# Autodesk Inventor assembly: OpenROV_Dev_Port_EndCap
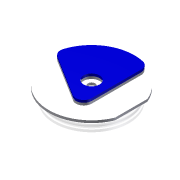
[picture p0: Inventor's stored thumbnail of the model, 180x180]
Saved by Autodesk Inventor 2012 (Build 160160000, 160)
## iProperties
Created: 2012-07-04
Part Number: OpenROV_Dev_Port_EndCap
Document SubType Name: Assembly
Designer: user
Author: user
## Documents named in this file (6)
- C:\Users\user\Desktop\CLEAN ME\OpenROV\openrov-hardware\OpenROV 2.3.2 Dev\OpenROV_Dev_Port_EndCap.iam
- C:\Users\user\Desktop\CLEAN ME\OpenROV\openrov-hardware\OpenROV 2.3.2 Dev\OpenROV_Dev_EndCap_90.ipt
- C:\Users\user\Desktop\CLEAN ME\OpenROV\openrov-hardware\OpenROV 2.3.2 Dev\OpenROV_Dev_EndCap_94.ipt
- C:\Users\user\Desktop\CLEAN ME\OpenROV\openrov-hardware\OpenROV 2.3.2 Dev\OpenROV_Dev_EndCap_108.ipt
- C:\Users\user\Desktop\CLEAN ME\OpenROV\openrov-hardware\OpenROV 2.3.2 Dev\OpenROV_Dev_EndCap_Wire_Guide.ipt
- C:\Users\user\Desktop\CLEAN ME\OpenROV\openrov-hardware\OpenROV 2.3.2 Dev\OpenROV_Dev_EndCap_Wire Guide_Cover.ipt
## Components (8 placed, 5 different names)
1. OpenROV_Dev_EndCap_90:1 — Mate:1, Mate:2, Mate:5, Mate:6, Mate:9, Mate:10
2. OpenROV_Dev_EndCap_90:2 — Mate:3, Mate:4, Mate:7, Mate:8, Mate:11, Mate:12
3. OpenROV_Dev_EndCap_94:1 — Mate:2, Mate:3, Mate:6, Mate:7, Mate:10, Mate:11
4. OpenROV_Dev_EndCap_94:2 — Mate:4, Mate:8, Mate:12, Mate:13, Mate:14, Mate:15
5. OpenROV_Dev_EndCap_94:3 — Mate:1, Mate:5, Mate:9
6. OpenROV_Dev_EndCap_108:1 — Mate:13, Mate:14, Mate:15, Mate:16, Mate:17, Mate:18
7. OpenROV_Dev_EndCap_Wire_Guide:1 — Mate:16, Mate:17, Mate:18, Mate:19, Mate:20, Flush:1
8. OpenROV_Dev_EndCap_Wire Guide_Cover:1 — Mate:19, Mate:20, Flush:1
## Relationships (21: Mate 20, Flush 1)
- Mate:1: OpenROV_Dev_EndCap_90:1 ↔ OpenROV_Dev_EndCap_94:3
- Mate:2: OpenROV_Dev_EndCap_90:1 ↔ OpenROV_Dev_EndCap_94:1
- Mate:3: OpenROV_Dev_EndCap_90:2 ↔ OpenROV_Dev_EndCap_94:1
- Mate:4: OpenROV_Dev_EndCap_90:2 ↔ OpenROV_Dev_EndCap_94:2
- Mate:5: OpenROV_Dev_EndCap_90:1 ↔ OpenROV_Dev_EndCap_94:3
- Mate:6: OpenROV_Dev_EndCap_90:1 ↔ OpenROV_Dev_EndCap_94:1
- Mate:7: OpenROV_Dev_EndCap_90:2 ↔ OpenROV_Dev_EndCap_94:1
- Mate:8: OpenROV_Dev_EndCap_90:2 ↔ OpenROV_Dev_EndCap_94:2
- Mate:9: OpenROV_Dev_EndCap_90:1 ↔ OpenROV_Dev_EndCap_94:3
- Mate:10: OpenROV_Dev_EndCap_90:1 ↔ OpenROV_Dev_EndCap_94:1
- Mate:11: OpenROV_Dev_EndCap_90:2 ↔ OpenROV_Dev_EndCap_94:1
- Mate:12: OpenROV_Dev_EndCap_90:2 ↔ OpenROV_Dev_EndCap_94:2
- Mate:13: OpenROV_Dev_EndCap_94:2 ↔ OpenROV_Dev_EndCap_108:1
- Mate:14: OpenROV_Dev_EndCap_94:2 ↔ OpenROV_Dev_EndCap_108:1
- Mate:15: OpenROV_Dev_EndCap_94:2 ↔ OpenROV_Dev_EndCap_108:1
- Mate:16: OpenROV_Dev_EndCap_108:1 ↔ OpenROV_Dev_EndCap_Wire_Guide:1
- Mate:17: OpenROV_Dev_EndCap_108:1 ↔ OpenROV_Dev_EndCap_Wire_Guide:1
- Mate:18: OpenROV_Dev_EndCap_108:1 ↔ OpenROV_Dev_EndCap_Wire_Guide:1
- Mate:19: OpenROV_Dev_EndCap_Wire_Guide:1 ↔ OpenROV_Dev_EndCap_Wire Guide_Cover:1
- Mate:20: OpenROV_Dev_EndCap_Wire_Guide:1 ↔ OpenROV_Dev_EndCap_Wire Guide_Cover:1
- Flush:1: OpenROV_Dev_EndCap_Wire_Guide:1 ↔ OpenROV_Dev_EndCap_Wire Guide_Cover:1
